# Autodesk Inventor assembly: Assembly1
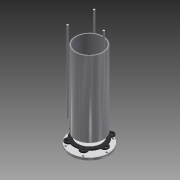
[picture p0: Inventor's stored thumbnail of the model, 180x180]
Saved by Autodesk Inventor 2015 (Build 190159000, 159)
## iProperties
Created: 2015-02-28
Part Number: Assembly1
Document SubType Name: Assembly
Designer: Qiuyang
Author: Qiuyang
## Documents named in this file (5)
- C:\Users\Qiuyang\Dropbox\VIP\SeaPerch\Dimensions\Aluminium_structure\Assembly1.iam
- C:\Users\Qiuyang\Dropbox\VIP\SeaPerch\Dimensions\Aluminium_structure\tube.ipt
- C:\Users\Qiuyang\Dropbox\VIP\SeaPerch\Dimensions\Aluminium_structure\rubber ring.ipt
- C:\Users\Qiuyang\Dropbox\VIP\SeaPerch\Dimensions\Aluminium_structure\cap.ipt
- C:\Users\Qiuyang\Dropbox\VIP\SeaPerch\Dimensions\Aluminium_structure\threaded rod.ipt
## Components (6 placed, 4 different names)
1. tube:1 — Insert:1, Insert:2
2. threaded rod:1
3. threaded rod:2
4. threaded rod:3
5. cap:1 — Insert:2
6. rubber ring:1 — Insert:1
## Relationships (2: Insert 2)
- Insert:1 (12.7 mm): tube:1 ↔ rubber ring:1
- Insert:2 (25.4 mm): tube:1 ↔ cap:1
